# Autodesk Inventor assembly: Assembly bottom改
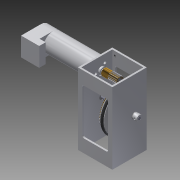
[picture p0: Inventor's stored thumbnail of the model, 180x180]
Saved by Autodesk Inventor 2015 (Build 190159000, 159)
## iProperties
Created: 2015-05-23
Part Number: Assembly bottom改
Document SubType Name: Assembly
Designer: kenta
Mass: 265.884 g
Surface Area: 636.789 cm^2
Volume: 87.1566 cm^3
Density: 3.05065 g/cm^3
Author: kenta
## Documents named in this file (11)
- C:\Users\kenta\Documents\Inventor\知能ロボコン\Assembly bottom ver2.iam
- C:\Users\kenta\Documents\Inventor\知能ロボコン\Shaft.ipt
- C:\Users\kenta\Documents\Inventor\知能ロボコン\Motor_A-max22.ipt
- C:\Users\kenta\Documents\Inventor\知能ロボコン\Bearing_SMF63ZZ.ipt
- C:\Users\kenta\Documents\Inventor\知能ロボコン\Wheel.ipt
- C:\Users\kenta\Documents\Inventor\知能ロボコン\Wheel ring.ipt
- C:\Users\kenta\Documents\Inventor\知能ロボコン\Stopper.ipt
- C:\Users\kenta\Documents\Inventor\知能ロボコン\Gear box ver2.ipt
- C:\Users\kenta\Documents\Inventor\知能ロボコン\Gear1_GEAB0.5-16-8-K-4.ipt
- C:\Users\kenta\Documents\Inventor\知能ロボコン\Gear2_S50B 90B+0203.ipt
- C:\Users\kenta\Documents\Inventor\知能ロボコン\Assembly bottom ver2\デザイン アクセラレータ\平歯車1.iam
## Components (14 placed, 10 different names)
1. Wheel:1 — 挿入:24, 挿入:28, メイト:1
2. Bearing_SMF63ZZ:3 — 挿入:19, 挿入:26, 挿入:29
3. Bearing_SMF63ZZ:4 — 挿入:9, 挿入:18, 挿入:27, 挿入:30
4. Shaft:2 — 挿入:9
5. Motor_A-max22:1 — 挿入:22, 挿入:23, 挿入:25, 挿入:31, 挿入:32
6. Stopper:3 — 挿入:18
7. Stopper:5 — 挿入:19
8. Gear box ver2:1 — 挿入:22, 挿入:23, 挿入:26, 挿入:27, 挿入:28
9. Gear1_GEAB0.5-16-8-K-4:1 — 挿入:25, メイト:3, フラッシュ:2, メイト:5, フラッシュ:4
10. Gear2_S50B 90B+0203:1 — 挿入:24, メイト:2, フラッシュ:1, メイト:4, フラッシュ:3
11. Wheel ring:1 — メイト:1
12. Gear box ver2:1 — 挿入:29, 挿入:30, 挿入:31, 挿入:32
13. 平歯車:1 [sub-assembly] — メイト:2, フラッシュ:1, メイト:3, フラッシュ:2
14. 平歯車:2 [sub-assembly] — メイト:4, フラッシュ:3, メイト:5, フラッシュ:4
## Relationships (23: Insert 14, Mate 5, Flush 4)
- 挿入:9 [Insert] (-5 mm): Bearing_SMF63ZZ:4 ↔ Shaft:2
- 挿入:18 [Insert]: Bearing_SMF63ZZ:4 ↔ Stopper:3
- 挿入:19 [Insert]: Bearing_SMF63ZZ:3 ↔ Stopper:5
- 挿入:22 [Insert]: Motor_A-max22:1 ↔ Gear box ver2:1
- 挿入:23 [Insert]: Motor_A-max22:1 ↔ Gear box ver2:1
- 挿入:24 [Insert]: Wheel:1 ↔ Gear2_S50B 90B+0203:1
- 挿入:25 [Insert] (-9 mm): Motor_A-max22:1 ↔ Gear1_GEAB0.5-16-8-K-4:1
- 挿入:26 [Insert]: Bearing_SMF63ZZ:3 ↔ Gear box ver2:1
- 挿入:27 [Insert]: Bearing_SMF63ZZ:4 ↔ Gear box ver2:1
- 挿入:28 [Insert] (9.5 mm): Wheel:1 ↔ Gear box ver2:1
- メイト:1 [Mate]: Wheel:1 ↔ Wheel ring:1
- 挿入:29 [Insert]: Bearing_SMF63ZZ:3 ↔ Gear box ver2:1
- 挿入:30 [Insert]: Bearing_SMF63ZZ:4 ↔ Gear box ver2:1
- 挿入:31 [Insert]: Motor_A-max22:1 ↔ Gear box ver2:1
- 挿入:32 [Insert]: Motor_A-max22:1 ↔ Gear box ver2:1
- メイト:2 [Mate]: Gear2_S50B 90B+0203:1 ↔ 平歯車:1
- フラッシュ:1 [Flush]: Gear2_S50B 90B+0203:1 ↔ 平歯車:1
- メイト:3 [Mate]: Gear1_GEAB0.5-16-8-K-4:1 ↔ 平歯車:1
- フラッシュ:2 [Flush]: Gear1_GEAB0.5-16-8-K-4:1 ↔ 平歯車:1
- メイト:4 [Mate]: Gear2_S50B 90B+0203:1 ↔ 平歯車:2
- フラッシュ:3 [Flush]: Gear2_S50B 90B+0203:1 ↔ 平歯車:2
- メイト:5 [Mate]: Gear1_GEAB0.5-16-8-K-4:1 ↔ 平歯車:2
- フラッシュ:4 [Flush]: Gear1_GEAB0.5-16-8-K-4:1 ↔ 平歯車:2
